# Autodesk Inventor assembly: Assembly1
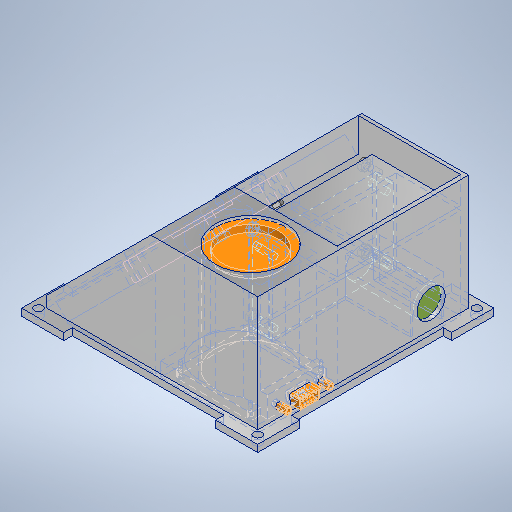
[picture p0: Inventor's stored thumbnail of the model, 512x512]
Saved by Autodesk Inventor 2025 (Build 290162000, 162)
## iProperties
Created: 2024-04-12
Part Number: Assembly1
Document SubType Name: Assembly
Designer: mahal
Author: mahal
## Documents named in this file (9)
- A:\study\IIST  COURSE\4th sem\MACHINING\project\Assembly1.iam
- A:\study\IIST  COURSE\4th sem\MACHINING\project\upper half second trial.ipt
- A:\study\IIST  COURSE\4th sem\MACHINING\project\sensor 1.ipt
- A:\study\IIST  COURSE\4th sem\MACHINING\project\sensor 2.ipt
- A:\study\IIST  COURSE\4th sem\MACHINING\project\sensor 3.ipt
- C:\Users\mahal\OneDrive\Documents\Inventor\Content Center Files\R2025\en-US\AS 1110\AS 1110 - M4 x 16.ipt
- C:\Users\mahal\OneDrive\Documents\Inventor\Content Center Files\R2025\en-US\AS 1110\AS 1110 - M4 x 10.ipt
- C:\Users\mahal\OneDrive\Documents\Inventor\Content Center Files\R2025\en-US\AS 1110\AS 1110 - M5 x 16.ipt
- C:\Users\mahal\OneDrive\Documents\Inventor\Content Center Files\R2025\en-US\UNI 6107\UNI 6107 - M2 x  8.ipt
## Components (15 placed, 8 different names)
1. upper half second trial:1 — Mate:1, Insert:1, Mate:2, Mate:3, Insert:2, Rotational:1, Insert:3, Insert:4, Insert:5, Insert:6, Insert:7
2. sensor 1:1 — Mate:1, Insert:1, Mate:2, Insert:11, Insert:12, Insert:13, Insert:14
3. sensor 2:1 — Mate:3, Insert:2
4. sensor 3:1 — Rotational:1, Insert:3, Insert:8, Insert:9, Insert:10
5. AS 1110 - Metric M4 x 10:1 — Insert:4
6. AS 1110 - Metric M4 x 10:2 — Insert:5
7. AS 1110 - Metric M4 x 10:3 — Insert:6
8. AS 1110 - Metric M4 x 10:4 — Insert:7
9. AS 1110 - Metric M5 x 16:1 — Insert:8
10. AS 1110 - Metric M4 x 16:1 — Insert:9
11. AS 1110 - Metric M4 x 16:2 — Insert:10
12. UNI 6107 M2 x  8:1 — Insert:11
13. UNI 6107 M2 x  8:2 — Insert:12
14. UNI 6107 M2 x  8:3 — Insert:13
15. UNI 6107 M2 x  8:4 — Insert:14
## Relationships (18: Insert 14, Mate 3, RevoluteJoint 1)
- Mate:1: upper half second trial:1 ↔ sensor 1:1
- Insert:1: upper half second trial:1 ↔ sensor 1:1
- Mate:2: upper half second trial:1 ↔ sensor 1:1
- Mate:3: upper half second trial:1 ↔ sensor 2:1
- Insert:2: upper half second trial:1 ↔ sensor 2:1
- Rotational:1 [RevoluteJoint]: upper half second trial:1 ↔ sensor 3:1
- Insert:3: upper half second trial:1 ↔ sensor 3:1
- Insert:4: upper half second trial:1 ↔ AS 1110 - Metric M4 x 10:1
- Insert:5: upper half second trial:1 ↔ AS 1110 - Metric M4 x 10:2
- Insert:6: upper half second trial:1 ↔ AS 1110 - Metric M4 x 10:3
- Insert:7: upper half second trial:1 ↔ AS 1110 - Metric M4 x 10:4
- Insert:8: sensor 3:1 ↔ AS 1110 - Metric M5 x 16:1
- Insert:9: sensor 3:1 ↔ AS 1110 - Metric M4 x 16:1
- Insert:10: sensor 3:1 ↔ AS 1110 - Metric M4 x 16:2
- Insert:11: sensor 1:1 ↔ UNI 6107 M2 x  8:1
- Insert:12: sensor 1:1 ↔ UNI 6107 M2 x  8:2
- Insert:13: sensor 1:1 ↔ UNI 6107 M2 x  8:3
- Insert:14: sensor 1:1 ↔ UNI 6107 M2 x  8:4
